# Autodesk Inventor assembly: body
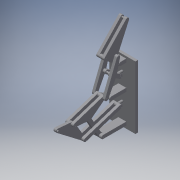
[picture p0: Inventor's stored thumbnail of the model, 180x180]
Saved by Autodesk Inventor 2016 (Build 200138000, 138)
## iProperties
Created: 2018-05-06
Part Number: body
Material: 一般
Document SubType Name: Assembly
Designer: 黃胤瑋
Author: 黃胤瑋
## Documents named in this file (19)
- C:\Users\黃胤瑋\Desktop\mechanism\Two stage six link lifting mechanism\body.iam
- C:\Users\黃胤瑋\Desktop\mechanism\Two stage six link lifting mechanism\實體1.ipt
- C:\Users\黃胤瑋\Desktop\mechanism\Two stage six link lifting mechanism\實體2.ipt
- C:\Users\黃胤瑋\Desktop\mechanism\Two stage six link lifting mechanism\實體3.ipt
- C:\Users\黃胤瑋\Desktop\mechanism\Two stage six link lifting mechanism\實體4.ipt
- C:\Users\黃胤瑋\Desktop\mechanism\Two stage six link lifting mechanism\實體5.ipt
- C:\Users\黃胤瑋\Desktop\mechanism\Two stage six link lifting mechanism\實體6.ipt
- C:\Users\黃胤瑋\Desktop\mechanism\Two stage six link lifting mechanism\實體7.ipt
- C:\Users\黃胤瑋\Desktop\mechanism\Two stage six link lifting mechanism\實體9.ipt
- C:\Users\黃胤瑋\Desktop\mechanism\Two stage six link lifting mechanism\實體10.ipt
- C:\Users\黃胤瑋\Desktop\mechanism\Two stage six link lifting mechanism\實體11.ipt
- C:\Users\黃胤瑋\Desktop\mechanism\Two stage six link lifting mechanism\實體12.ipt
- C:\Users\黃胤瑋\Desktop\mechanism\Two stage six link lifting mechanism\實體13.ipt
- C:\Users\黃胤瑋\Desktop\mechanism\Two stage six link lifting mechanism\實體14.ipt
- C:\Users\黃胤瑋\Desktop\mechanism\Two stage six link lifting mechanism\實體15.ipt
- C:\Users\黃胤瑋\Desktop\mechanism\Two stage six link lifting mechanism\實體16.ipt
- C:\Users\黃胤瑋\Desktop\mechanism\Two stage six link lifting mechanism\銷6.ipt
- C:\Users\黃胤瑋\Desktop\mechanism\Two stage six link lifting mechanism\銷9.ipt
- C:\Users\黃胤瑋\Desktop\mechanism\Two stage six link lifting mechanism\銷12.ipt
## Components (29 placed, 18 different names)
1. 實體1:1
2. 實體2:1
3. 實體3:1
4. 實體4:1
5. 實體5:1 — 貼合:12, 齊平:8, 貼合:13, 齊平:9
6. 實體6:1
7. 實體7:1 — 貼合:14, 齊平:10, 貼合:16, 齊平:12
8. 實體9:1 — 貼合:7, 齊平:7, 貼合:18
9. 實體10:1 — 貼合:2
10. 實體11:1 — 齊平:3
11. 實體12:1 — 齊平:2, 貼合:3
12. 實體13:1 — 貼合:4, 齊平:4, 貼合:17, 齊平:13
13. 實體14:1 — 貼合:5, 齊平:5, 齊平:14
14. 實體15:1
15. 實體16:1 — 貼合:6, 齊平:6, 貼合:10, 貼合:11, 貼合:15, 齊平:11
16. 銷6:1 — 貼合:3, 齊平:3
17. 銷9:1 — 貼合:2, 齊平:2
18. 銷9:2 — 貼合:5, 齊平:5
19. 銷9:3 — 貼合:6, 齊平:6
20. 銷9:4 — 貼合:13, 齊平:9
21. 銷9:6 — 貼合:12, 齊平:8
22. 銷9:7 — 貼合:7, 齊平:7
23. 銷9:8 — 貼合:10, 貼合:11
24. 銷12:5 — 貼合:4, 齊平:4
25. 銷9:9 — 貼合:14, 齊平:10
26. 銷9:10 — 貼合:15, 齊平:11
27. 銷9:11 — 貼合:16, 齊平:12
28. 銷12:6 — 貼合:17, 齊平:13
29. 銷12:7 — 貼合:18, 齊平:14
## Relationships (28: Mate 15, Flush 13)
- 貼合:2 [Mate]: 實體10:1 ↔ 銷9:1
- 齊平:2 [Flush]: 實體12:1 ↔ 銷9:1
- 貼合:3 [Mate]: 實體12:1 ↔ 銷6:1
- 齊平:3 [Flush]: 實體11:1 ↔ 銷6:1
- 貼合:4 [Mate]: 實體13:1 ↔ 銷12:5
- 齊平:4 [Flush]: 實體13:1 ↔ 銷12:5
- 貼合:5 [Mate]: 實體14:1 ↔ 銷9:2
- 齊平:5 [Flush]: 實體14:1 ↔ 銷9:2
- 貼合:6 [Mate]: 實體16:1 ↔ 銷9:3
- 齊平:6 [Flush]: 實體16:1 ↔ 銷9:3
- 貼合:7 [Mate]: 實體9:1 ↔ 銷9:7
- 齊平:7 [Flush]: 實體9:1 ↔ 銷9:7
- 貼合:10 [Mate]: 實體16:1 ↔ 銷9:8
- 貼合:11 [Mate]: 實體16:1 ↔ 銷9:8
- 貼合:12 [Mate]: 實體5:1 ↔ 銷9:6
- 齊平:8 [Flush]: 實體5:1 ↔ 銷9:6
- 貼合:13 [Mate]: 實體5:1 ↔ 銷9:4
- 齊平:9 [Flush]: 實體5:1 ↔ 銷9:4
- 貼合:14 [Mate]: 實體7:1 ↔ 銷9:9
- 齊平:10 [Flush]: 實體7:1 ↔ 銷9:9
- 貼合:15 [Mate]: 實體16:1 ↔ 銷9:10
- 齊平:11 [Flush]: 實體16:1 ↔ 銷9:10
- 貼合:16 [Mate]: 實體7:1 ↔ 銷9:11
- 齊平:12 [Flush]: 實體7:1 ↔ 銷9:11
- 貼合:17 [Mate]: 實體13:1 ↔ 銷12:6
- 齊平:13 [Flush]: 實體13:1 ↔ 銷12:6
- 貼合:18 [Mate]: 實體9:1 ↔ 銷12:7
- 齊平:14 [Flush]: 實體14:1 ↔ 銷12:7
